# Autodesk Inventor assembly: Assembly
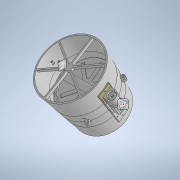
[picture p0: Inventor's stored thumbnail of the model, 180x180]
Saved by Autodesk Inventor 2020.2 (Build 242310000, 310)
## iProperties
Created: 2020-04-21
Part Number: Assembly
Document SubType Name: Assembly
Designer: Josiah
Author: Josiah
## Documents named in this file (8)
- C:\Users\josia\OneDrive\Apps\0011_VentControlValve\Drawings\Assembly.iam
- C:\Users\josia\OneDrive\Apps\0011_VentControlValve\Drawings\Base.ipt
- C:\Users\josia\OneDrive\Apps\0011_VentControlValve\Drawings\Butterfly Valve.ipt
- C:\Users\josia\OneDrive\Apps\0011_VentControlValve\Drawings\Center Section - Back.ipt
- C:\Users\josia\OneDrive\Apps\0011_VentControlValve\Drawings\Center Section - Front.ipt
- C:\Users\josia\OneDrive\Apps\0011_VentControlValve\Drawings\limitSwitch.ipt
- C:\Users\josia\OneDrive\Apps\0011_VentControlValve\Drawings\motor+Gearbox.ipt
- C:\Users\josia\OneDrive\Apps\0011_VentControlValve\Drawings\MotorBracket.ipt
## Components (9 placed, 7 different names)
1. Base:1 — Mate:6, Mate:7, Mate:8
2. Butterfly Valve:1 — Rotational:1, Mate:12
3. Center Section - Back:1 — Mate:1, Mate:2, Mate:3, Mate:4, Mate:5, Rotational:1, Mate:9, Mate:10, Mate:11, Mate:13, Mate:14, Mate:15, Mate:16, Mate:17
4. Center Section - Front:1 — Mate:1, Mate:2, Mate:6, Mate:7, Mate:8, Mate:18, Mate:19, Mate:20
5. limitSwitch:1 — Mate:18, Mate:19, Mate:20
6. motor+Gearbox:1 — Mate:12, Mate:13, Mate:14
7. MotorBracket:1 — Mate:9, Mate:10, Mate:11
8. Base:2 — Mate:3, Mate:4, Mate:5
9. limitSwitch:2 — Mate:15, Mate:16, Mate:17
## Relationships (21: Mate 20, RevoluteJoint 1)
- Mate:1: Center Section - Back:1 ↔ Center Section - Front:1
- Mate:2: Center Section - Back:1 ↔ Center Section - Front:1
- Mate:3: Center Section - Back:1 ↔ Base:2
- Mate:4: Center Section - Back:1 ↔ Base:2
- Mate:5: Center Section - Back:1 ↔ Base:2
- Mate:6: Base:1 ↔ Center Section - Front:1
- Mate:7: Base:1 ↔ Center Section - Front:1
- Mate:8: Base:1 ↔ Center Section - Front:1
- Rotational:1 [RevoluteJoint]: Butterfly Valve:1 ↔ Center Section - Back:1
- Mate:9: Center Section - Back:1 ↔ MotorBracket:1
- Mate:10: Center Section - Back:1 ↔ MotorBracket:1
- Mate:11: Center Section - Back:1 ↔ MotorBracket:1
- Mate:12: Butterfly Valve:1 ↔ motor+Gearbox:1
- Mate:13: Center Section - Back:1 ↔ motor+Gearbox:1
- Mate:14: Center Section - Back:1 ↔ motor+Gearbox:1
- Mate:15: Center Section - Back:1 ↔ limitSwitch:2
- Mate:16: Center Section - Back:1 ↔ limitSwitch:2
- Mate:17 (0.2 mm): Center Section - Back:1 ↔ limitSwitch:2
- Mate:18: Center Section - Front:1 ↔ limitSwitch:1
- Mate:19: Center Section - Front:1 ↔ limitSwitch:1
- Mate:20 (0.2 mm): Center Section - Front:1 ↔ limitSwitch:1
